# Autodesk Inventor assembly: Magnet Frame for 4040 - Assembly
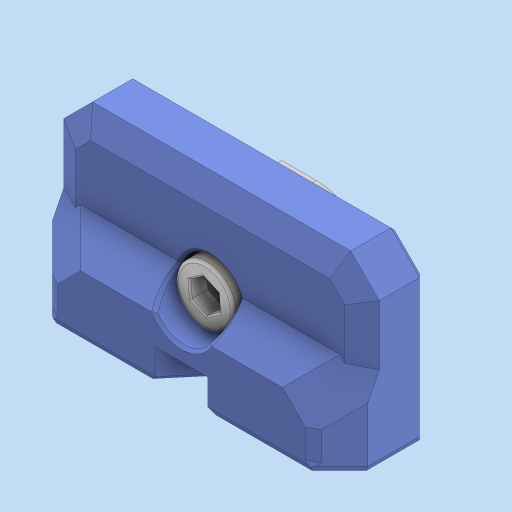
[picture p0: Inventor's stored thumbnail of the model, 512x512]
Saved by Autodesk Inventor 2023.2 (Build 272271000, 271)
## iProperties
Created: 2023-11-29
Part Number: Magnet Frame for 4040 - Assembly
Document SubType Name: Assembly
Designer: Nils Bade
Author: Nils Bade
## Documents named in this file (5)
- C:\Users\nilsb\Documents\Inventor\Projektarbeit-Bade\Enclosure\Magnet Frame for 4040 - Assembly.iam
- C:\Users\nilsb\Documents\Inventor\Projektarbeit-Bade\Enclosure\Magnet Frame 90deg for 4040.ipt
- C:\Users\nilsb\Documents\Inventor\Projektarbeit-Bade\Enclosure\Magnet-RatrigEnclosure.ipt
- C:\Users\nilsb\Documents\Inventor\Projektarbeit-Bade\Schrauben\Cap Head Screw M6x16.ipt
- C:\Users\nilsb\Documents\Inventor\Projektarbeit-Bade\RatRig_modified\T-NUT - DropIn 4040 SERIES - M6.ipt
## Components (5 placed, 4 different names)
1. Magnet Frame 90deg for 4040:1 — Passend:1, Passend:2, Passend:3, Passend:4, Passend:7, Passend:8
2. Magnet-RatrigEnclosure:1 — Passend:1, Passend:3
3. Magnet-RatrigEnclosure:2 — Passend:2, Passend:4
4. T-NUT - DROP IN TYPE FOR 40 SERIES - M6:1
5. Cap Head Screw M6x16:1 — Passend:7, Passend:8
## Relationships (9: Mate 8, Angle 1)
- Passend:1 [Mate]: Magnet Frame 90deg for 4040:1 ↔ Magnet-RatrigEnclosure:1
- Passend:2 [Mate]: Magnet Frame 90deg for 4040:1 ↔ Magnet-RatrigEnclosure:2
- Passend:3 [Mate]: Magnet Frame 90deg for 4040:1 ↔ Magnet-RatrigEnclosure:1
- Passend:4 [Mate]: Magnet Frame 90deg for 4040:1 ↔ Magnet-RatrigEnclosure:2
- [Mate]: Magnet Frame 90deg for 4040:1 ↔ T-NUT - DROP IN TYPE FOR 40 SERIES - M6:1
- [Angle] (0 deg): Magnet Frame 90deg for 4040:1 ↔ T-NUT - DROP IN TYPE FOR 40 SERIES - M6:1
- [Mate] (4.5 mm): Magnet Frame 90deg for 4040:1 ↔ T-NUT - DROP IN TYPE FOR 40 SERIES - M6:1
- Passend:7 [Mate]: Magnet Frame 90deg for 4040:1 ↔ Cap Head Screw M6x16:1
- Passend:8 [Mate]: Magnet Frame 90deg for 4040:1 ↔ Cap Head Screw M6x16:1
